# Autodesk Inventor assembly: c1
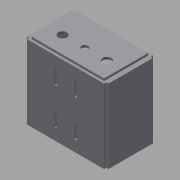
[picture p0: Inventor's stored thumbnail of the model, 180x180]
Saved by Autodesk Inventor 2016 (Build 200138000, 138)
## iProperties
Created: 2015-10-11
Part Number: c1
Document SubType Name: Assembly
Designer: daniel
Author: daniel
## Documents named in this file (8)
- C:\Users\daniel\Documents\GitHub\cardboard-stage-metric\stage\c1.iam
- C:\Users\daniel\Documents\GitHub\cardboard-stage-metric\stage\c1a.ipt
- C:\Users\daniel\Documents\GitHub\cardboard-stage-metric\stage\c1b.ipt
- C:\Users\daniel\Documents\GitHub\cardboard-stage-metric\stage\c1c.ipt
- C:\Users\daniel\Documents\GitHub\cardboard-stage-metric\stage\c1d.ipt
- C:\Users\daniel\Documents\GitHub\cardboard-stage-metric\stage\c1e.ipt
- C:\Users\daniel\Documents\GitHub\cardboard-stage-metric\stage\c1f.ipt
- C:\Users\daniel\Documents\GitHub\cardboard-stage-metric\stage\c1h.ipt
## Components (13 placed, 7 different names)
1. c1a:1 — Mate:3, Mate:4, Flush:1, Flush:2, Mate:5, Mate:8, Mate:9, Mate:17, Mate:18
2. c1b:1 — Mate:5, Mate:6, Mate:19, Mate:20, Mate:21, Flush:16
3. c1c:1 — Mate:8, Mate:9, Flush:14, Flush:17, Flush:18, Mate:23, Mate:24, Mate:25, Mate:26
4. c1d:1 — Mate:4, Flush:2, Mate:6, Flush:7, Mate:13, Mate:17, Mate:22, Mate:27
5. c1e:1 — Flush:5, Flush:6, Flush:7, Mate:11, Mate:12, Mate:14, Mate:15, Flush:10
6. c1f:1 — Flush:8, Flush:9, Mate:14, Mate:15, Flush:10
7. c1d:2 — Mate:3, Flush:1, Mate:11, Mate:12, Mate:18
8. c1e:2 — Flush:5, Flush:6, Mate:13, Mate:16
9. c1f:2 — Flush:8, Flush:9, Mate:16
10. c1h:1 — Flush:18, Mate:24, Mate:25, Mate:27
11. c1h:2 — Flush:13, Flush:15, Mate:21, Flush:16, Mate:22
12. c1h:3 — Flush:13, Flush:14, Mate:19, Flush:15, Mate:20
13. c1h:4 — Flush:17, Mate:23, Mate:26
## Relationships (37: Mate 23, Flush 14)
- Mate:3: c1a:1 ↔ c1d:2
- Mate:4: c1a:1 ↔ c1d:1
- Flush:1: c1a:1 ↔ c1d:2
- Flush:2: c1a:1 ↔ c1d:1
- Mate:5: c1a:1 ↔ c1b:1
- Mate:6: c1b:1 ↔ c1d:1
- Mate:8: c1a:1 ↔ c1c:1
- Mate:9: c1a:1 ↔ c1c:1
- Flush:5: c1e:1 ↔ c1e:2
- Flush:6: c1e:1 ↔ c1e:2
- Flush:7: c1d:1 ↔ c1e:1
- Mate:11: c1e:1 ↔ c1d:2
- Mate:12: c1e:1 ↔ c1d:2
- Mate:13: c1d:1 ↔ c1e:2
- Flush:8: c1f:1 ↔ c1f:2
- Flush:9: c1f:1 ↔ c1f:2
- Mate:14: c1e:1 ↔ c1f:1
- Mate:15: c1e:1 ↔ c1f:1
- Flush:10: c1e:1 ↔ c1f:1
- Mate:16: c1e:2 ↔ c1f:2
- Flush:13: c1h:2 ↔ c1h:3
- Mate:17: c1a:1 ↔ c1d:1
- Mate:18: c1a:1 ↔ c1d:2
- Flush:14: c1c:1 ↔ c1h:3
- Mate:19: c1b:1 ↔ c1h:3
- Flush:15: c1h:2 ↔ c1h:3
- Mate:20: c1b:1 ↔ c1h:3
- Mate:21: c1b:1 ↔ c1h:2
- Flush:16: c1b:1 ↔ c1h:2
- Mate:22: c1d:1 ↔ c1h:2
- Flush:17: c1c:1 ↔ c1h:4
- Flush:18: c1c:1 ↔ c1h:1
- Mate:23: c1c:1 ↔ c1h:4
- Mate:24: c1c:1 ↔ c1h:1
- Mate:25: c1c:1 ↔ c1h:1
- Mate:26: c1c:1 ↔ c1h:4
- Mate:27: c1d:1 ↔ c1h:1
